# Autodesk Inventor assembly: Frame
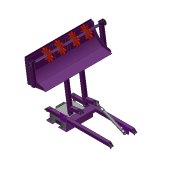
[picture p0: Inventor's stored thumbnail of the model, 180x180]
Saved by Autodesk Inventor 2012 (Build 160160000, 160)
## iProperties
Created: 2013-01-19
Part Number: Frame
Document SubType Name: Assembly
Designer: JesseK
Mass: 10203.8 g
Surface Area: 16729.5 cm^2
Volume: 3587.64 cm^3
Density: 2.84414 g/cm^3
Author: JesseK
## Documents named in this file (15)
- Z:\UserData\Documents\Inventor\team1885frc\Robot2013\FloorPickup\Frame.iam
- Z:\UserData\Documents\Inventor\team1885frc\Robot2013\FrontRearRail.ipt
- Z:\UserData\Documents\Inventor\team1885frc\Robot2013\SpatulaPivotMount.ipt
- Z:\UserData\Documents\Inventor\team1885frc\Pneumatics\046-DXP_6inStrokex075Bore\046_DXP_R_D_129__F_D_166_3_.iam
- Z:\UserData\Documents\Inventor\team1885frc\Robot2013\FloorPickup\ShovelAssembly.iam
- Z:\UserData\Documents\Inventor\team1885frc\Electronics\Battery.ipt
- Z:\UserData\Documents\Inventor\team1885frc\Robot2013\FloorPickup\Shovel_PivotMount.ipt
- Z:\UserData\Documents\Inventor\team1885frc\Hardware\Bolts\Bolt_0.25_20_1.25len_SocketHead.ipt
- Z:\UserData\Documents\Inventor\team1885frc\Hardware\Nuts\LockNut_0.25_20.ipt
- Z:\UserData\Documents\Inventor\team1885frc\Hardware\Bolts\Bolt_0.25_20_1.75len_SocketHead.ipt
- Z:\UserData\Documents\Inventor\team1885frc\Robot2013\FloorPickup\Shovel_CylinderMountSpacer.ipt
- Z:\UserData\Documents\Inventor\team1885frc\Robot2013\FloorPickup\BatteryMount.ipt
- Z:\UserData\Documents\Inventor\team1885frc\Robot2013\FloorPickup\BatteryStandoff.ipt
- Z:\UserData\Documents\Inventor\team1885frc\Hardware\Bolts\Bolt_0.25_20_0.75len_SocketHead.ipt
- Z:\UserData\Documents\Inventor\team1885frc\Hardware\Bolts\Bolt_0.25_20_3.0len_SocketHead.ipt
## Components (39 placed, 14 different names)
1. FrontRearRail:1 — Mate:2, Flush:1, Mate:6, Mate:53, Mate:58, Flush:9, Mate:61, Mate:64, Mate:102, Mate:103, Mate:104, Mate:105, Mate:117, Mate:120, Mate:122, Mate:123
2. FrontRearRail:2 — Mate:4, Mate:5, Mate:6, Mate:17, Flush:6, Mate:54, Flush:7, Flush:8, Mate:100, Mate:101, Mate:106, Mate:107, Mate:108, Mate:118, Mate:119, Mate:121, Mate:124
3. SpatulaPivotMount:1 — Mate:2, Flush:1, Mate:4, Mate:5, Mate:17, Mate:55, Mate:82, Flush:10
4. 046-DXP:1 [sub-assembly] — Mate:51, Mate:78, Mate:81, Mate:132
5. ShovelAssembly:1 [sub-assembly] — Mate:51, Mate:53, Mate:56, Mate:67, Mate:68, Mate:69, Mate:70, Mate:72, Mate:74, Mate:125, Mate:126, Mate:127, Mate:128
6. Battery:1 — Flush:6, Mate:54, Mate:99
7. Shovel_PivotMount:1 — Flush:7, Mate:55, Flush:8, Mate:56, Mate:65, Mate:66
8. Shovel_PivotMount:2 — Mate:64, Mate:65, Mate:66
9. Shovel_PivotMount:3 — Mate:58, Flush:9, Mate:61, Mate:77, Mate:80, Mate:131
10. Bolt_0.25_20_1.25len_SocketHead:1 — Mate:69, Mate:70, Mate:73
11. Bolt_0.25_20_1.25len_SocketHead:2 — Mate:67, Mate:68, Mate:71
12. LockNut_0.25_20:1 — Mate:71, Mate:72
13. LockNut_0.25_20:2 — Mate:73, Mate:74
14. LockNut_0.25_20:3 — Mate:76, Mate:77
15. Bolt_0.25_20_1.75len_SocketHead:1 — Mate:76, Mate:78, Mate:79, Mate:131, Mate:132
16. Shovel_CylinderMountSpacer:1 — Mate:79, Mate:80, Mate:81
17. BatteryMount:1 — Mate:82, Flush:10, Mate:83, Mate:84, Mate:85, Mate:86, Mate:87, Mate:88, Mate:89, Mate:90, Mate:91, Mate:92, Mate:93, Mate:94, Mate:95, Mate:96, Mate:97, Mate:98, Mate:99, Mate:108, Mate:109, Mate:110, Mate:111, Mate:112
18. BatteryStandoff:1 — Mate:83, Mate:84
19. BatteryStandoff:2 — Mate:85, Mate:86
20. BatteryStandoff:3 — Mate:87, Mate:88
21. BatteryStandoff:4 — Mate:89, Mate:90
22. Bolt_0.25_20_0.75len_SocketHead:1 — Mate:94, Mate:97
23. Bolt_0.25_20_0.75len_SocketHead:2 — Mate:95, Mate:98
24. Bolt_0.25_20_0.75len_SocketHead:3 — Mate:93, Mate:96
25. Bolt_0.25_20_0.75len_SocketHead:4 — Mate:91, Mate:92
26. Bolt_0.25_20_0.75len_SocketHead:5 — Mate:103, Mate:104
27. Bolt_0.25_20_0.75len_SocketHead:6 — Mate:102, Mate:105
28. Bolt_0.25_20_0.75len_SocketHead:7 — Mate:101, Mate:106
29. Bolt_0.25_20_0.75len_SocketHead:8 — Mate:100, Mate:107
30. Bolt_0.25_20_0.75len_SocketHead:9 — Mate:110, Mate:111
31. Bolt_0.25_20_0.75len_SocketHead:10 — Mate:109, Mate:112
32. Bolt_0.25_20_0.75len_SocketHead:11 — Mate:118, Mate:119
33. Bolt_0.25_20_0.75len_SocketHead:12 — Mate:117, Mate:120
34. Bolt_0.25_20_0.75len_SocketHead:13 — Mate:122, Mate:123
35. Bolt_0.25_20_0.75len_SocketHead:14 — Mate:121, Mate:124
36. Bolt_0.25_20_3.0len_SocketHead:1 — Mate:125, Mate:128, Mate:130, Flush:12
37. Bolt_0.25_20_3.0len_SocketHead:2 — Mate:126, Mate:127, Mate:129, Flush:11
38. LockNut_0.25_20:4 — Mate:129, Flush:11
39. LockNut_0.25_20:5 — Mate:130, Flush:12
## Relationships (84: Mate 76, Flush 8)
- Mate:2: FrontRearRail:1 ↔ SpatulaPivotMount:1
- Flush:1: FrontRearRail:1 ↔ SpatulaPivotMount:1
- Mate:4: FrontRearRail:2 ↔ SpatulaPivotMount:1
- Mate:5: FrontRearRail:2 ↔ SpatulaPivotMount:1
- Mate:6: FrontRearRail:1 ↔ FrontRearRail:2
- Mate:17 (203.2 mm): FrontRearRail:2 ↔ SpatulaPivotMount:1
- Mate:51: 046-DXP:1 ↔ ShovelAssembly:1
- Mate:53 (12.7 mm): FrontRearRail:1 ↔ ShovelAssembly:1
- Flush:6 (25.4 mm): FrontRearRail:2 ↔ Battery:1
- Mate:54: FrontRearRail:2 ↔ Battery:1
- Flush:7: FrontRearRail:2 ↔ Shovel_PivotMount:1
- Mate:55: SpatulaPivotMount:1 ↔ Shovel_PivotMount:1
- Flush:8: FrontRearRail:2 ↔ Shovel_PivotMount:1
- Mate:56: ShovelAssembly:1 ↔ Shovel_PivotMount:1
- Mate:58: FrontRearRail:1 ↔ Shovel_PivotMount:3
- Flush:9: FrontRearRail:1 ↔ Shovel_PivotMount:3
- Mate:61 (50.8 mm): FrontRearRail:1 ↔ Shovel_PivotMount:3
- Mate:64: FrontRearRail:1 ↔ Shovel_PivotMount:2
- Mate:65: Shovel_PivotMount:1 ↔ Shovel_PivotMount:2
- Mate:66: Shovel_PivotMount:1 ↔ Shovel_PivotMount:2
- Mate:67: ShovelAssembly:1 ↔ Bolt_0.25_20_1.25len_SocketHead:2
- Mate:68: ShovelAssembly:1 ↔ Bolt_0.25_20_1.25len_SocketHead:2
- Mate:69: ShovelAssembly:1 ↔ Bolt_0.25_20_1.25len_SocketHead:1
- Mate:70: ShovelAssembly:1 ↔ Bolt_0.25_20_1.25len_SocketHead:1
- Mate:71: Bolt_0.25_20_1.25len_SocketHead:2 ↔ LockNut_0.25_20:1
- Mate:72: ShovelAssembly:1 ↔ LockNut_0.25_20:1
- Mate:73: Bolt_0.25_20_1.25len_SocketHead:1 ↔ LockNut_0.25_20:2
- Mate:74: ShovelAssembly:1 ↔ LockNut_0.25_20:2
- Mate:76: LockNut_0.25_20:3 ↔ Bolt_0.25_20_1.75len_SocketHead:1
- Mate:77: Shovel_PivotMount:3 ↔ LockNut_0.25_20:3
- Mate:78: 046-DXP:1 ↔ Bolt_0.25_20_1.75len_SocketHead:1
- Mate:79: Bolt_0.25_20_1.75len_SocketHead:1 ↔ Shovel_CylinderMountSpacer:1
- Mate:80: Shovel_PivotMount:3 ↔ Shovel_CylinderMountSpacer:1
- Mate:81: 046-DXP:1 ↔ Shovel_CylinderMountSpacer:1
- Mate:82: SpatulaPivotMount:1 ↔ BatteryMount:1
- Flush:10: SpatulaPivotMount:1 ↔ BatteryMount:1
- Mate:83: BatteryMount:1 ↔ BatteryStandoff:1
- Mate:84: BatteryMount:1 ↔ BatteryStandoff:1
- Mate:85: BatteryMount:1 ↔ BatteryStandoff:2
- Mate:86: BatteryMount:1 ↔ BatteryStandoff:2
- Mate:87: BatteryMount:1 ↔ BatteryStandoff:3
- Mate:88: BatteryMount:1 ↔ BatteryStandoff:3
- Mate:89: BatteryMount:1 ↔ BatteryStandoff:4
- Mate:90: BatteryMount:1 ↔ BatteryStandoff:4
- Mate:91: BatteryMount:1 ↔ Bolt_0.25_20_0.75len_SocketHead:4
- Mate:92: BatteryMount:1 ↔ Bolt_0.25_20_0.75len_SocketHead:4
- Mate:93: BatteryMount:1 ↔ Bolt_0.25_20_0.75len_SocketHead:3
- Mate:94: BatteryMount:1 ↔ Bolt_0.25_20_0.75len_SocketHead:1
- Mate:95: BatteryMount:1 ↔ Bolt_0.25_20_0.75len_SocketHead:2
- Mate:96: BatteryMount:1 ↔ Bolt_0.25_20_0.75len_SocketHead:3
- Mate:97: BatteryMount:1 ↔ Bolt_0.25_20_0.75len_SocketHead:1
- Mate:98: BatteryMount:1 ↔ Bolt_0.25_20_0.75len_SocketHead:2
- Mate:99: Battery:1 ↔ BatteryMount:1
- Mate:100: FrontRearRail:2 ↔ Bolt_0.25_20_0.75len_SocketHead:8
- Mate:101: FrontRearRail:2 ↔ Bolt_0.25_20_0.75len_SocketHead:7
- Mate:102: FrontRearRail:1 ↔ Bolt_0.25_20_0.75len_SocketHead:6
- Mate:103: FrontRearRail:1 ↔ Bolt_0.25_20_0.75len_SocketHead:5
- Mate:104: FrontRearRail:1 ↔ Bolt_0.25_20_0.75len_SocketHead:5
- Mate:105: FrontRearRail:1 ↔ Bolt_0.25_20_0.75len_SocketHead:6
- Mate:106: FrontRearRail:2 ↔ Bolt_0.25_20_0.75len_SocketHead:7
- Mate:107: FrontRearRail:2 ↔ Bolt_0.25_20_0.75len_SocketHead:8
- Mate:108 (6.35 mm): FrontRearRail:2 ↔ BatteryMount:1
- Mate:109: BatteryMount:1 ↔ Bolt_0.25_20_0.75len_SocketHead:10
- Mate:110: BatteryMount:1 ↔ Bolt_0.25_20_0.75len_SocketHead:9
- Mate:111: BatteryMount:1 ↔ Bolt_0.25_20_0.75len_SocketHead:9
- Mate:112: BatteryMount:1 ↔ Bolt_0.25_20_0.75len_SocketHead:10
- Mate:117: FrontRearRail:1 ↔ Bolt_0.25_20_0.75len_SocketHead:12
- Mate:118: FrontRearRail:2 ↔ Bolt_0.25_20_0.75len_SocketHead:11
- Mate:119: FrontRearRail:2 ↔ Bolt_0.25_20_0.75len_SocketHead:11
- Mate:120: FrontRearRail:1 ↔ Bolt_0.25_20_0.75len_SocketHead:12
- Mate:121: FrontRearRail:2 ↔ Bolt_0.25_20_0.75len_SocketHead:14
- Mate:122: FrontRearRail:1 ↔ Bolt_0.25_20_0.75len_SocketHead:13
- Mate:123: FrontRearRail:1 ↔ Bolt_0.25_20_0.75len_SocketHead:13
- Mate:124: FrontRearRail:2 ↔ Bolt_0.25_20_0.75len_SocketHead:14
- Mate:125: ShovelAssembly:1 ↔ Bolt_0.25_20_3.0len_SocketHead:1
- Mate:126: ShovelAssembly:1 ↔ Bolt_0.25_20_3.0len_SocketHead:2
- Mate:127: ShovelAssembly:1 ↔ Bolt_0.25_20_3.0len_SocketHead:2
- Mate:128: ShovelAssembly:1 ↔ Bolt_0.25_20_3.0len_SocketHead:1
- Mate:129: Bolt_0.25_20_3.0len_SocketHead:2 ↔ LockNut_0.25_20:4
- Flush:11: Bolt_0.25_20_3.0len_SocketHead:2 ↔ LockNut_0.25_20:4
- Mate:130: Bolt_0.25_20_3.0len_SocketHead:1 ↔ LockNut_0.25_20:5
- Flush:12: Bolt_0.25_20_3.0len_SocketHead:1 ↔ LockNut_0.25_20:5
- Mate:131: Shovel_PivotMount:3 ↔ Bolt_0.25_20_1.75len_SocketHead:1
- Mate:132: 046-DXP:1 ↔ Bolt_0.25_20_1.75len_SocketHead:1
